# Autodesk Inventor assembly: CameraAssembly
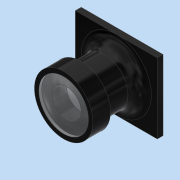
[picture p0: Inventor's stored thumbnail of the model, 180x180]
Saved by Autodesk Inventor 2017 (Build 210142000, 142)
## iProperties
Created: 2018-02-22
Part Number: CameraAssembly
Document SubType Name: Assembly
Designer: Derek Wider
Author: Derek Wider
## Documents named in this file (3)
- G:\Projects\Submarine\Submarine-project\CAD\midships\Sail\camera\CameraAssembly.iam
- G:\Projects\Submarine\Submarine-project\CAD\midships\Sail\camera\Camera.ipt
- G:\Projects\Submarine\Submarine-project\CAD\midships\Sail\camera\Lense.ipt
## Components (2 placed, 2 different names)
1. Camera:1 — Mate:1, Mate:2
2. Lense:1 — Mate:1, Mate:2
## Relationships (2: Mate 2)
- Mate:1: Camera:1 ↔ Lense:1
- Mate:2: Camera:1 ↔ Lense:1
